# Autodesk Inventor assembly: scara
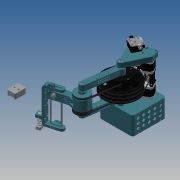
[picture p0: Inventor's stored thumbnail of the model, 180x180]
Saved by Autodesk Inventor 2013 (Build 170138000, 138)
## iProperties
Created: 2017-03-31
Part Number: scara
Document SubType Name: Assembly
Designer: employee
Author: employee
## Documents named in this file (53)
- C:\Users\employee\Desktop\SCARA\scara.iam
- C:\Users\employee\Desktop\SCARA\top plate.ipt
- C:\Users\employee\Desktop\SCARA\stepper.ipt
- C:\Users\employee\Desktop\SCARA\dual stepper mount.ipt
- C:\Users\employee\Desktop\SCARA\washer.ipt
- C:\Users\employee\Desktop\SCARA\drive pulley.ipt
- C:\Users\employee\Desktop\SCARA\608 bearing.ipt
- C:\Users\employee\Desktop\SCARA\offset shield.ipt
- C:\Users\employee\Desktop\SCARA\M3x30.ipt
- C:\Users\employee\Desktop\SCARA\235 drive pulley.ipt
- C:\Users\employee\Desktop\SCARA\M3x60.ipt
- C:\Users\employee\Desktop\SCARA\M3x35.ipt
- C:\Users\employee\Desktop\SCARA\M3x8.ipt
- C:\Users\employee\Desktop\SCARA\bottom plate.ipt
- C:\Users\employee\Desktop\SCARA\distal idler pulley.ipt
- C:\Users\employee\Desktop\SCARA\z idler pulley.ipt
- C:\Users\employee\Desktop\SCARA\central pivot spacer.ipt
- C:\Users\employee\Desktop\SCARA\distal drive pulley.ipt
- C:\Users\employee\Desktop\SCARA\lm6luu.ipt
- C:\Users\employee\Desktop\SCARA\rod.ipt
- C:\Users\employee\Desktop\SCARA\slide frame.ipt
- C:\Users\employee\Desktop\SCARA\heat block.ipt
- C:\Users\employee\Desktop\SCARA\heat sink.ipt
- C:\Users\employee\Desktop\SCARA\nozzle.ipt
- C:\Users\employee\Desktop\SCARA\e3d mount.ipt
- C:\Users\employee\Desktop\SCARA\M3x45.ipt
- C:\Users\employee\Desktop\SCARA\M3x65.ipt
- C:\Users\employee\Desktop\SCARA\Imported Components\175_filament_feed\175_filament_feed.ipt
- C:\Users\employee\Desktop\SCARA\Imported Components\big_gear\big_gear.ipt
- C:\Users\employee\Desktop\SCARA\Imported Components\cilindar_fitting\cilindar_fitting.ipt
- C:\Users\employee\Desktop\SCARA\Imported Components\e3d extruder\e3d extruder.ipt
- C:\Users\employee\Desktop\SCARA\Imported Components\gornji dio e3d extruder\gornji dio e3d extruder.ipt
- C:\Users\employee\Desktop\SCARA\Imported Components\polugica\polugica.ipt
- C:\Users\employee\Desktop\SCARA\Imported Components\small gear\small gear.ipt
- C:\Users\employee\Desktop\SCARA\M3x25.ipt
- C:\Users\employee\Desktop\SCARA\first belt.ipt
- C:\Users\employee\Desktop\SCARA\middle belt.ipt
- C:\Users\employee\Desktop\SCARA\belt tensioner.ipt
- C:\Users\employee\Desktop\SCARA\M8x120.ipt
- C:\Users\employee\Desktop\SCARA\M8x200.ipt
- C:\Users\employee\Desktop\SCARA\M3 nut.ipt
- C:\Users\employee\Desktop\SCARA\z idler pulley 3.ipt
- C:\Users\employee\Desktop\SCARA\distal arm 2.ipt
- C:\Users\employee\Desktop\SCARA\distal arm end.ipt
- C:\Users\employee\Desktop\SCARA\driven arm 2_1.ipt
- C:\Users\employee\Desktop\SCARA\driven arm2_2.ipt
- C:\Users\employee\Desktop\SCARA\thin arm 2_1.ipt
- C:\Users\employee\Desktop\SCARA\thin arm2_2.ipt
- C:\Users\employee\Desktop\SCARA\m5 washer.ipt
- C:\Users\employee\Desktop\SCARA\f605zz.ipt
- C:\Users\employee\Desktop\SCARA\M5x40 BHCS.ipt
- C:\Users\employee\Desktop\SCARA\bottom plate cap.ipt
- C:\Users\employee\Desktop\SCARA\wire block.ipt
## Components (131 placed, 52 different names)
1. stepper:1 — Insert:2, Insert:3, Insert:7, Insert:8, Angle:2, Mate:14
2. stepper:2 — Insert:1, Insert:4, Insert:5, Insert:6, Insert:15
3. dual stepper mount:1 — Insert:5, Insert:6, Insert:12, Insert:13, Flush:1, Insert:28, Insert:29, Insert:30, Insert:34, Insert:35, Insert:36
4. dual stepper mount:2 — Insert:7, Insert:8, Insert:10, Insert:11, Insert:31, Insert:32, Insert:33, Insert:37, Insert:38, Insert:39
5. washer:1 — Insert:9, Insert:17
6. stepper:3 — Insert:10, Insert:11, Mate:1, Insert:41, Mate:17
7. stepper:4 — Insert:12, Insert:13, Insert:14, Insert:40
8. drive pulley:1 — Flush:1, Mate:1
9. drive pulley:2 — Insert:15, Mate:19
10. drive pulley:3 — Insert:14, Mate:18
11. 608 bearing:2 — Insert:17, Insert:150
12. offset shield:1 — Insert:20, Insert:25, Insert:26, Insert:27, Insert:46, Insert:47, Mate:28, Mate:29
13. 608 bearing:3 — Insert:20, Insert:21
14. washer:2 — Insert:21, Insert:44
15. M3x30:1 — Insert:148
16. 235 drive pulley:1 — Insert:46, Insert:47, Insert:111
17. M3x60:1 — Insert:149, Mate:28
18. M3x35:1 — Insert:25
19. M3x35:2 — Insert:26
20. M3x35:3 — Insert:27
21. M3x8:1 — Insert:33
22. M3x8:2 — Insert:28
23. M3x8:3 — Insert:29
24. M3x8:4 — Insert:31
25. M3x8:5 — Insert:32
26. M3x8:6 — Insert:30
27. M3x8:7 — Insert:36
28. M3x8:8 — Insert:35
29. M3x8:9 — Insert:34
30. M3x8:10 — Insert:37
31. M3x8:11 — Insert:38
32. M3x8:12 — Insert:39
33. bottom plate:1 — Insert:40, Insert:41, Insert:89, Insert:90, Insert:91, Insert:92, Insert:93, Insert:94, Insert:95, Insert:96, z, y, x, Insert:153, Insert:165, Insert:166
34. distal idler pulley:1 — Insert:42, Insert:43, Insert:112, Insert:115
35. 608 bearing:4 — Insert:42, Insert:44
36. 608 bearing:5 — Insert:43, Insert:45
37. washer:3 — Insert:45, Insert:50
38. z idler pulley:2 — Insert:48, Insert:49, Insert:113, Insert:114
39. 608 bearing:6 — Insert:48, Insert:51
40. 608 bearing:7 — Insert:49, Insert:50
41. washer:4 — Insert:51, Insert:54
42. 608 bearing:8 — Insert:54
43. 608 bearing:9 — Insert:55, Insert:156
44. washer:5 — Insert:55, Insert:88
45. central pivot spacer:1 — Insert:88, Insert:153
46. washer:6 — Insert:62, Insert:152
47. washer:7 — Insert:143
48. distal drive pulley:1 — Insert:61, Insert:66, Insert:67, Insert:68, Insert:69, Mate:26, Insert:145
49. 608 bearing:10 — Insert:61, Insert:62
50. M3x30:2 — Insert:66
51. M3x30:3 — Insert:67
52. M3x30:4 — Insert:68, Mate:33
53. M3x30:5 — Insert:69
54. lm6luu:1 — Mate:4, Insert:146
55. lm6luu:2 — Mate:5, Insert:147
56. rod:1 — Mate:5, Insert:83
57. rod:2 — Mate:4, Insert:82
58. slide frame:1 — Insert:82, Insert:83, Angle:1, Mate:11, Flush:3, Mate:13, Flush:5, Mate:24, Mate:25, Insert:123, Insert:124, Insert:135, Insert:136, Insert:137, Insert:138, Insert:139, Insert:140, Angle:9, Angle:10, Angle:11, Angle:12, Angle:13, Angle:14
59. heat block:1 — Insert:84, Angle:15
60. heat sink:1 — Insert:84, Insert:85, Mate:8, Mate:9, Mate:12
61. nozzle:1 — Insert:85, z, y, x
62. e3d mount:1 — Mate:8, Mate:10, Mate:11, Flush:3, Mate:13
63. e3d mount:2 — Mate:9, Mate:10, Angle:1, Mate:12, Insert:86, Insert:87, Angle:15
64. M3x30:6 — Insert:86
65. M3x30:7 — Insert:87
66. M3x45:1 — Insert:96
67. M3x45:2 — Insert:95
68. M3x45:3 — Insert:93
69. M3x45:4 — Insert:91
70. M3x45:5 — Insert:90
71. M3x45:6 — Insert:89
72. M3x45:7 — Insert:92
73. M3x45:8 — Insert:94
74. M3x65:1 — Insert:97
75. M3x65:2 — Insert:99
76. M3x65:3 — Insert:100
77. M3x65:4 — Insert:98
78. 175_filament_feed:1 — Insert:102, Angle:3
79. big_gear:1 — Insert:105
80. cilindar_fitting:1 — Insert:103
81. e3d extruder:1 — Insert:101, Angle:2, Insert:102, Angle:3, Mate:15, Angle:4, Insert:103, Insert:105, Insert:106, Angle:5, Insert:167
82. gornji dio e3d extruder:1 — Insert:106, Angle:5, Insert:107, Insert:108, Insert:109, Insert:110
83. polugica:1 — Mate:14, Mate:16, Insert:104
84. small gear:1 — Insert:104
85. M3x35:4 — Insert:107
86. M3x35:5 — Insert:108
87. M3x35:6 — Insert:109
88. M3x25:1 — Insert:110
89. first belt:1 — Insert:111, Mate:19
90. first belt:2 — Insert:112, Mate:17
91. first belt:3 — Insert:113, Mate:18
92. middle belt:1 — Insert:114, Mate:32
93. middle belt:2 — Insert:115, Mate:26
94. belt tensioner:3 — Insert:119, Insert:120, Mate:25, Insert:127, Insert:128
95. belt tensioner:4 — Insert:119, Insert:120, Flush:5, Mate:24
96. belt tensioner:5 — Insert:121, Insert:122, Insert:123, Insert:124
97. belt tensioner:6 — Insert:121, Insert:122, Insert:125, Insert:126
98. M3x35:7 — Insert:125
99. M3x35:8 — Insert:126
100. M3x35:9 — Insert:127
101. M3x35:10 — Insert:128
102. M8x120:1 — Insert:151, Mate:31
103. M8x200:1 — Insert:129
104. M3 nut:1 — Insert:135, Angle:14
105. M3 nut:2 — Insert:140, Angle:9
106. M3 nut:3 — Insert:139, Angle:10
107. M3 nut:4 — Insert:138, Angle:11
108. M3 nut:5 — Insert:137, Angle:12
109. M3 nut:6 — Insert:136, Angle:13
110. z idler pulley 3:1 — Insert:141, Insert:142
111. 608 bearing:11 — Insert:141, Insert:143
112. 608 bearing:12 — Insert:142, Insert:144
113. washer:8 — Insert:144, Insert:155
114. distal arm 2:1 — Insert:145, Flush:6, Flush:7, Mate:27, Insert:154, Mate:33
115. distal arm end:1 — Flush:6, Flush:7, Mate:27, Insert:146, Insert:147, Insert:157, Insert:158
116. driven arm 2_1:1 — Insert:148, Insert:149, Insert:150, Mate:29, Flush:8, Flush:9, Mate:30
117. driven arm2_2:1 — Flush:8, Flush:9, Mate:30, Insert:151, Insert:152
118. 608 bearing:13 — Insert:154, Insert:155
119. thin arm 2_1:1 — Insert:156, Flush:10, Flush:11
120. thin arm2_2:1 — Flush:10, Flush:11, Mate:31, Mate:32
121. m5 washer:1 — Insert:157, Insert:159
122. m5 washer:2 — Insert:158, Insert:162
123. f605zz:1 — Insert:160, Insert:161
124. f605zz:2 — Insert:159, Insert:160
125. f605zz:3 — Insert:163, Insert:164
126. f605zz:4 — Insert:162, Insert:163
127. M5x40 BHCS:1 — Insert:161
128. M5x40 BHCS:2 — Insert:164
129. bottom plate cap:1 — Insert:165, Insert:166
130. wire block:1
131. top plate:1 — Insert:1, Insert:2, Insert:3, Insert:4, Insert:9, Insert:97, Insert:98, Insert:99, Insert:100, Insert:101, Insert:129, Insert:167
## Relationships (180: Insert 131, Mate 27, Angle 12, Flush 10)
- Insert:1: stepper:2 ↔ top plate:1
- Insert:2: stepper:1 ↔ top plate:1
- Insert:3: stepper:1 ↔ top plate:1
- Insert:4: stepper:2 ↔ top plate:1
- Insert:5: stepper:2 ↔ dual stepper mount:1
- Insert:6: stepper:2 ↔ dual stepper mount:1
- Insert:7: stepper:1 ↔ dual stepper mount:2
- Insert:8: stepper:1 ↔ dual stepper mount:2
- Insert:9: washer:1 ↔ top plate:1
- Insert:10: dual stepper mount:2 ↔ stepper:3
- Insert:11: dual stepper mount:2 ↔ stepper:3
- Insert:12: dual stepper mount:1 ↔ stepper:4
- Insert:13: dual stepper mount:1 ↔ stepper:4
- Insert:14 (3.75 mm): stepper:4 ↔ drive pulley:3
- Insert:15 (3.5 mm): stepper:2 ↔ drive pulley:2
- Flush:1: dual stepper mount:1 ↔ drive pulley:1
- Mate:1: stepper:3 ↔ drive pulley:1
- Insert:17: washer:1 ↔ 608 bearing:2
- Insert:20: offset shield:1 ↔ 608 bearing:3
- Insert:21: 608 bearing:3 ↔ washer:2
- Insert:25: offset shield:1 ↔ M3x35:1
- Insert:26: offset shield:1 ↔ M3x35:2
- Insert:27: offset shield:1 ↔ M3x35:3
- Insert:28: dual stepper mount:1 ↔ M3x8:2
- Insert:29: dual stepper mount:1 ↔ M3x8:3
- Insert:30: dual stepper mount:1 ↔ M3x8:6
- Insert:31: dual stepper mount:2 ↔ M3x8:4
- Insert:32: dual stepper mount:2 ↔ M3x8:5
- Insert:33: dual stepper mount:2 ↔ M3x8:1
- Insert:34: dual stepper mount:1 ↔ M3x8:9
- Insert:35: dual stepper mount:1 ↔ M3x8:8
- Insert:36: dual stepper mount:1 ↔ M3x8:7
- Insert:37: dual stepper mount:2 ↔ M3x8:10
- Insert:38: dual stepper mount:2 ↔ M3x8:11
- Insert:39: dual stepper mount:2 ↔ M3x8:12
- Insert:40: stepper:4 ↔ bottom plate:1
- Insert:41: stepper:3 ↔ bottom plate:1
- Insert:42: distal idler pulley:1 ↔ 608 bearing:4
- Insert:43: distal idler pulley:1 ↔ 608 bearing:5
- Insert:44: washer:2 ↔ 608 bearing:4
- Insert:45: 608 bearing:5 ↔ washer:3
- Insert:46: offset shield:1 ↔ 235 drive pulley:1
- Insert:47: offset shield:1 ↔ 235 drive pulley:1
- Insert:48: z idler pulley:2 ↔ 608 bearing:6
- Insert:49: z idler pulley:2 ↔ 608 bearing:7
- Insert:50: washer:3 ↔ 608 bearing:7
- Insert:51: 608 bearing:6 ↔ washer:4
- Insert:54: washer:4 ↔ 608 bearing:8
- Insert:55: 608 bearing:9 ↔ washer:5
- Insert:61: distal drive pulley:1 ↔ 608 bearing:10
- Insert:62: washer:6 ↔ 608 bearing:10
- Insert:66: distal drive pulley:1 ↔ M3x30:2
- Insert:67: distal drive pulley:1 ↔ M3x30:3
- Insert:68: distal drive pulley:1 ↔ M3x30:4
- Insert:69: distal drive pulley:1 ↔ M3x30:5
- Mate:4: lm6luu:1 ↔ rod:2
- Mate:5: lm6luu:2 ↔ rod:1
- Insert:82: rod:2 ↔ slide frame:1
- Insert:83: rod:1 ↔ slide frame:1
- Insert:84: heat block:1 ↔ heat sink:1
- Insert:85: heat sink:1 ↔ nozzle:1
- Mate:8: heat sink:1 ↔ e3d mount:1
- Mate:9: heat sink:1 ↔ e3d mount:2
- Mate:10: e3d mount:1 ↔ e3d mount:2
- Angle:1 (0 deg): slide frame:1 ↔ e3d mount:2
- Mate:11: slide frame:1 ↔ e3d mount:1
- Flush:3: slide frame:1 ↔ e3d mount:1
- Mate:12: heat sink:1 ↔ e3d mount:2
- Mate:13: slide frame:1 ↔ e3d mount:1
- Insert:86: e3d mount:2 ↔ M3x30:6
- Insert:87: e3d mount:2 ↔ M3x30:7
- Insert:88: washer:5 ↔ central pivot spacer:1
- Insert:89: bottom plate:1 ↔ M3x45:6
- Insert:90: bottom plate:1 ↔ M3x45:5
- Insert:91: bottom plate:1 ↔ M3x45:4
- Insert:92: bottom plate:1 ↔ M3x45:7
- Insert:93: bottom plate:1 ↔ M3x45:3
- Insert:94: bottom plate:1 ↔ M3x45:8
- Insert:95: bottom plate:1 ↔ M3x45:2
- Insert:96: bottom plate:1 ↔ M3x45:1
- Insert:97: M3x65:1 ↔ top plate:1
- Insert:98: M3x65:4 ↔ top plate:1
- Insert:99: M3x65:2 ↔ top plate:1
- Insert:100: M3x65:3 ↔ top plate:1
- Insert:101: e3d extruder:1 ↔ top plate:1
- Angle:2 (0 deg): stepper:1 ↔ e3d extruder:1
- Insert:102: 175_filament_feed:1 ↔ e3d extruder:1
- Angle:3 (0 deg): 175_filament_feed:1 ↔ e3d extruder:1
- Mate:14: stepper:1 ↔ polugica:1
- Mate:15: e3d extruder:1
- Angle:4 (0 deg): e3d extruder:1
- Mate:16: polugica:1
- Insert:103: cilindar_fitting:1 ↔ e3d extruder:1
- Insert:104: polugica:1 ↔ small gear:1
- Insert:105: big_gear:1 ↔ e3d extruder:1
- Insert:106: e3d extruder:1 ↔ gornji dio e3d extruder:1
- Angle:5 (0 deg): e3d extruder:1 ↔ gornji dio e3d extruder:1
- Insert:107: gornji dio e3d extruder:1 ↔ M3x35:4
- Insert:108: gornji dio e3d extruder:1 ↔ M3x35:5
- Insert:109: gornji dio e3d extruder:1 ↔ M3x35:6
- Insert:110: gornji dio e3d extruder:1 ↔ M3x25:1
- Insert:111 (1 mm): 235 drive pulley:1 ↔ first belt:1
- Insert:112 (1 mm): distal idler pulley:1 ↔ first belt:2
- Insert:113 (1 mm): z idler pulley:2 ↔ first belt:3
- Mate:17: stepper:3 ↔ first belt:2
- Mate:18: drive pulley:3 ↔ first belt:3
- Mate:19: drive pulley:2 ↔ first belt:1
- Insert:114 (1 mm): z idler pulley:2 ↔ middle belt:1
- Insert:115 (1 mm): distal idler pulley:1 ↔ middle belt:2
- z [Flush] (-10 mm): bottom plate:1 ↔ nozzle:1
- y [Mate] (79 mm): bottom plate:1 ↔ nozzle:1
- x [Mate]: bottom plate:1 ↔ nozzle:1
- Insert:119: belt tensioner:3 ↔ belt tensioner:4
- Insert:120: belt tensioner:3 ↔ belt tensioner:4
- Flush:5: slide frame:1 ↔ belt tensioner:4
- Mate:24: slide frame:1 ↔ belt tensioner:4
- Mate:25: slide frame:1 ↔ belt tensioner:3
- Insert:121: belt tensioner:5 ↔ belt tensioner:6
- Insert:122: belt tensioner:5 ↔ belt tensioner:6
- Insert:123: slide frame:1 ↔ belt tensioner:5
- Insert:124: slide frame:1 ↔ belt tensioner:5
- Insert:125: belt tensioner:6 ↔ M3x35:7
- Insert:126: belt tensioner:6 ↔ M3x35:8
- Insert:127: belt tensioner:3 ↔ M3x35:9
- Insert:128: belt tensioner:3 ↔ M3x35:10
- Insert:129: M8x200:1 ↔ top plate:1
- Insert:135: slide frame:1 ↔ M3 nut:1
- Insert:136: slide frame:1 ↔ M3 nut:6
- Insert:137: slide frame:1 ↔ M3 nut:5
- Insert:138: slide frame:1 ↔ M3 nut:4
- Insert:139: slide frame:1 ↔ M3 nut:3
- Insert:140: slide frame:1 ↔ M3 nut:2
- Angle:9 (0 deg): slide frame:1 ↔ M3 nut:2
- Angle:10 (0 deg): slide frame:1 ↔ M3 nut:3
- Angle:11 (0 deg): slide frame:1 ↔ M3 nut:4
- Angle:12 (0 deg): slide frame:1 ↔ M3 nut:5
- Angle:13 (0 deg): slide frame:1 ↔ M3 nut:6
- Angle:14 (0 deg): slide frame:1 ↔ M3 nut:1
- Insert:141: z idler pulley 3:1 ↔ 608 bearing:11
- Insert:142: z idler pulley 3:1 ↔ 608 bearing:12
- Insert:143: washer:7 ↔ 608 bearing:11
- Insert:144: 608 bearing:12 ↔ washer:8
- Mate:26: distal drive pulley:1 ↔ middle belt:2
- Insert:145: distal drive pulley:1 ↔ distal arm 2:1
- Flush:6: distal arm 2:1 ↔ distal arm end:1
- Flush:7: distal arm 2:1 ↔ distal arm end:1
- Mate:27: distal arm 2:1 ↔ distal arm end:1
- Insert:146 (-2 mm): lm6luu:1 ↔ distal arm end:1
- Insert:147 (-2 mm): lm6luu:2 ↔ distal arm end:1
- Insert:148: M3x30:1 ↔ driven arm 2_1:1
- Insert:149: M3x60:1 ↔ driven arm 2_1:1
- Insert:150: 608 bearing:2 ↔ driven arm 2_1:1
- Mate:28: offset shield:1 ↔ M3x60:1
- Mate:29: offset shield:1 ↔ driven arm 2_1:1
- Flush:8: driven arm 2_1:1 ↔ driven arm2_2:1
- Flush:9: driven arm 2_1:1 ↔ driven arm2_2:1
- Mate:30: driven arm 2_1:1 ↔ driven arm2_2:1
- Insert:151: M8x120:1 ↔ driven arm2_2:1
- Insert:152: washer:6 ↔ driven arm2_2:1
- Insert:153: bottom plate:1 ↔ central pivot spacer:1
- Insert:154: distal arm 2:1 ↔ 608 bearing:13
- Insert:155: washer:8 ↔ 608 bearing:13
- Insert:156: 608 bearing:9 ↔ thin arm 2_1:1
- Flush:10: thin arm 2_1:1 ↔ thin arm2_2:1
- Flush:11: thin arm 2_1:1 ↔ thin arm2_2:1
- Mate:31: M8x120:1 ↔ thin arm2_2:1
- Mate:32: middle belt:1 ↔ thin arm2_2:1
- Insert:157: distal arm end:1 ↔ m5 washer:1
- Insert:158: distal arm end:1 ↔ m5 washer:2
- Insert:159: m5 washer:1 ↔ f605zz:2
- Insert:160: f605zz:1 ↔ f605zz:2
- Insert:161: f605zz:1 ↔ M5x40 BHCS:1
- Insert:162: m5 washer:2 ↔ f605zz:4
- Insert:163: f605zz:3 ↔ f605zz:4
- Insert:164: f605zz:3 ↔ M5x40 BHCS:2
- Mate:33: M3x30:4 ↔ distal arm 2:1
- Insert:165: bottom plate:1 ↔ bottom plate cap:1
- Insert:166: bottom plate:1 ↔ bottom plate cap:1
- Insert:167: e3d extruder:1 ↔ top plate:1
- Angle:15 (0 deg): heat block:1 ↔ e3d mount:2
## Named parameters: z = 10 mm, x = 75 mm, y = 100 mm
